# Autodesk Inventor assembly: Test_Electronics_Assembly
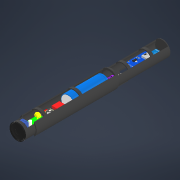
[picture p0: Inventor's stored thumbnail of the model, 180x180]
Saved by Autodesk Inventor 2022 (Build 260153000, 153)
## iProperties
Created: 2024-05-09
Part Number: Test_Electronics_Assembly
Document SubType Name: Assembly
Designer: jo_ki
Author: jo_ki
## Documents named in this file (13)
- C:\LocalRepos\Lightsaber Git\CAD\LightSaber_Inventor_Project\Assemblies\Electronics_Assembly.iam
- C:\LocalRepos\Lightsaber Git\CAD\LightSaber_Inventor_Project\Parts\Electronics_Housing.ipt
- C:\LocalRepos\Lightsaber Git\CAD\LightSaber_Inventor_Project\Import\ESP-WROOM32\ESP-WROOM32.iam
- C:\LocalRepos\Lightsaber Git\CAD\LightSaber_Inventor_Project\Import\Li-Ion-26650\26650.ipt
- C:\LocalRepos\Lightsaber Git\CAD\LightSaber_Inventor_Project\Parts\Electrical\Speaker_28mm.ipt
- C:\LocalRepos\Lightsaber Git\CAD\LightSaber_Inventor_Project\Import\lm386-mini-micro-audio-amplifier-module-1.snapshot.12\lm386gf.iam
- C:\LocalRepos\Lightsaber Git\CAD\LightSaber_Inventor_Project\Import\esp32-c3-supermini-1.snapshot.2\ESP32-C3 supermini v5.iam
- C:\LocalRepos\Lightsaber Git\CAD\LightSaber_Inventor_Project\Parts\Electrical\Boost-Buck-Converter.ipt
- C:\LocalRepos\Lightsaber Git\CAD\LightSaber_Inventor_Project\Import\sd-card-reader-4.snapshot.4\MicroSD Card Module - 2.iam
- C:\LocalRepos\Lightsaber Git\CAD\LightSaber_Inventor_Project\Import\logic-level-converter-5v-to-3-3v-module-1.snapshot.1\Logi Level Converter.iam
- C:\LocalRepos\Lightsaber Git\CAD\LightSaber_Inventor_Project\Import\bmi160-imu-1.snapshot.2\bmi160 v1.ipt
- C:\LocalRepos\Lightsaber Git\CAD\LightSaber_Inventor_Project\Import\push_buttons\A06-7.7\A06-7.7.ipt
- C:\LocalRepos\Lightsaber Git\CAD\LightSaber_Inventor_Project\Parts\Norm\Magnet_5x1mm.ipt
## Components (13 placed, 12 different names)
1. Test_Electronics_ Housing:1 — Mate:2, Mate:3, Mate:4, Mate:5, Mate:6, Mate:7, Mate:8, Mate:9
2. ESP-WROOM32:1 [sub-assembly]
3. 26650:1 — Mate:2
4. Speaker_28mm:1 — Mate:3, Mate:4
5. lm386gf:1 [sub-assembly]
6. ESP32-C3 supermini v5:1 [sub-assembly]
7. Boost-Buck-Converter:1
8. MicroSD Card Module - 2:1 [sub-assembly]
9. Logi Level Converter:1 [sub-assembly]
10. bmi160 v1:1
11. A06-7.7:1 — Mate:6, Flush:1
12. A06-7.7:2 — Mate:5, Mate:7, Flush:1
13. Magnet_5x1mm:1 — Mate:8, Mate:9
## Relationships (9: Mate 8, Flush 1)
- Mate:2: Test_Electronics_ Housing:1 ↔ 26650:1
- Mate:3: Test_Electronics_ Housing:1 ↔ Speaker_28mm:1
- Mate:4: Test_Electronics_ Housing:1 ↔ Speaker_28mm:1
- Mate:5: Test_Electronics_ Housing:1 ↔ A06-7.7:2
- Mate:6: Test_Electronics_ Housing:1 ↔ A06-7.7:1
- Mate:7 (-16 mm): Test_Electronics_ Housing:1 ↔ A06-7.7:2
- Flush:1: A06-7.7:1 ↔ A06-7.7:2
- Mate:8: Test_Electronics_ Housing:1 ↔ Magnet_5x1mm:1
- Mate:9: Test_Electronics_ Housing:1 ↔ Magnet_5x1mm:1
